# Autodesk Inventor assembly: antana
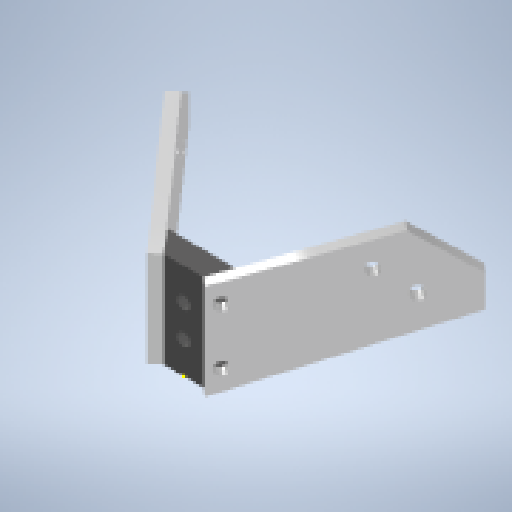
[picture p0: Inventor's stored thumbnail of the model, 512x512]
Saved by Autodesk Inventor 2026.1 (Build 301233020, 233B)
## iProperties
Created: 2024-02-25
Part Number: antana
Document SubType Name: Assembly
Designer: hibik
Author: hibik
## Documents named in this file (3)
- C:\Users\hibik\Documents\Robomech\HR\Eglantyne_mark2\hard\head\antana.iam
- C:\Users\hibik\Documents\Robomech\HR\Eglantyne_mark2\hard\head\antana_middle.ipt
- C:\Users\hibik\Documents\Robomech\HR\Eglantyne_mark2\hard\head\antana_side.ipt
## Components (3 placed, 2 different names)
1. antana_middle:1 — メイト:1, メイト:2, メイト:3, メイト:4, メイト:5, メイト:6
2. antana_side:1 — メイト:1, メイト:3, メイト:5
3. antana_side:2 — メイト:2, メイト:4, メイト:6
## Relationships (6: Mate 6)
- メイト:1 [Mate]: antana_middle:1 ↔ antana_side:1
- メイト:2 [Mate]: antana_middle:1 ↔ antana_side:2
- メイト:3 [Mate]: antana_middle:1 ↔ antana_side:1
- メイト:4 [Mate]: antana_middle:1 ↔ antana_side:2
- メイト:5 [Mate]: antana_middle:1 ↔ antana_side:1
- メイト:6 [Mate]: antana_middle:1 ↔ antana_side:2
